# Autodesk Inventor assembly: Сборка2
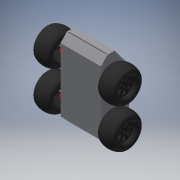
[picture p0: Inventor's stored thumbnail of the model, 180x180]
Saved by Autodesk Inventor 2019 (Build 230136000, 136)
## iProperties
Created: 2022-02-24
Part Number: Сборка2
Material: Типовые
Document SubType Name: Assembly
Designer: korsh
Author: korsh
## Documents named in this file (11)
- C:\Users\korsh\Desktop\Новая папка (7)\Сборка2.iam
- C:\Users\korsh\Desktop\Новая папка (7)\Моторный блок.iam
- C:\Users\korsh\Desktop\Новая папка (7)\боковина.ipt
- C:\Users\korsh\Desktop\Новая папка (7)\дно.ipt
- C:\Users\korsh\Desktop\Новая папка (7)\маленькое дно1.ipt
- C:\Users\korsh\Desktop\Новая папка (7)\мальенькое дно 2.ipt
- C:\Users\korsh\Desktop\Новая папка (7)\Деталь7.ipt
- C:\Users\korsh\Desktop\Новая папка (7)\задняя.ipt
- C:\Users\korsh\Desktop\Новая папка (7)\полуверх.ipt
- C:\Users\korsh\Desktop\Новая папка (7)\полуверх 2.ipt
- C:\Users\korsh\Desktop\Новая папка (7)\верх.ipt
## Components (14 placed, 10 different names)
1. Моторный блок:1 [sub-assembly] — Заподлицо:1, Заподлицо:2, Совмещение:1
2. Моторный блок:2 [sub-assembly] — Заподлицо:1, Заподлицо:2, Совмещение:1, Совмещение:2
3. боковина:1 — Совмещение:2, Заподлицо:3, Заподлицо:4, Совмещение:7, Заподлицо:6, Заподлицо:8, Совмещение:9, Заподлицо:12, Заподлицо:13, Заподлицо:17
4. боковина:2 — Заподлицо:3, Заподлицо:4, Совмещение:3, Совмещение:4, Совмещение:5, Совмещение:6, Совмещение:7, Заподлицо:5, Заподлицо:7, Заподлицо:9, Заподлицо:10, Заподлицо:11, Совмещение:8, Заподлицо:14, Заподлицо:15, Заподлицо:16
5. Моторный блок:3 [sub-assembly] — Совмещение:3, Совмещение:5
6. Моторный блок:4 [sub-assembly] — Совмещение:4, Совмещение:6
7. дно:1 — Заподлицо:5
8. маленькое дно1:1 — Заподлицо:6
9. мальенькое дно 2:1 — Заподлицо:7
10. лицо — Заподлицо:8, Совмещение:9, Заподлицо:12, Заподлицо:13
11. задняя:1 — Заподлицо:9, Заподлицо:10, Заподлицо:11, Совмещение:8
12. полуверх:1 — Заподлицо:14
13. полуверх 2:1 — Заподлицо:15, Заподлицо:16
14. верх:1 — Заподлицо:17
## Relationships (26: Flush 17, Mate 9)
- Заподлицо:1 [Flush]: Моторный блок:1 ↔ Моторный блок:2
- Заподлицо:2 [Flush]: Моторный блок:1 ↔ Моторный блок:2
- Совмещение:1 [Mate] (171 mm): Моторный блок:1 ↔ Моторный блок:2
- Совмещение:2 [Mate]: Моторный блок:2 ↔ боковина:1
- Заподлицо:3 [Flush]: боковина:1 ↔ боковина:2
- Заподлицо:4 [Flush]: боковина:1 ↔ боковина:2
- Совмещение:3 [Mate]: боковина:2 ↔ Моторный блок:3
- Совмещение:4 [Mate]: боковина:2 ↔ Моторный блок:4
- Совмещение:5 [Mate]: боковина:2 ↔ Моторный блок:3
- Совмещение:6 [Mate]: боковина:2 ↔ Моторный блок:4
- Совмещение:7 [Mate] (180 mm): боковина:1 ↔ боковина:2
- Заподлицо:5 [Flush]: боковина:2 ↔ дно:1
- Заподлицо:6 [Flush]: боковина:1 ↔ маленькое дно1:1
- Заподлицо:7 [Flush]: боковина:2 ↔ мальенькое дно 2:1
- Заподлицо:8 [Flush]: боковина:1 ↔ лицо
- Заподлицо:9 [Flush]: боковина:2 ↔ задняя:1
- Заподлицо:10 [Flush]: боковина:2 ↔ задняя:1
- Заподлицо:11 [Flush]: боковина:2 ↔ задняя:1
- Совмещение:8 [Mate]: боковина:2 ↔ задняя:1
- Совмещение:9 [Mate]: боковина:1 ↔ лицо
- Заподлицо:12 [Flush]: боковина:1 ↔ лицо
- Заподлицо:13 [Flush]: боковина:1 ↔ лицо
- Заподлицо:14 [Flush]: боковина:2 ↔ полуверх:1
- Заподлицо:15 [Flush]: боковина:2 ↔ полуверх 2:1
- Заподлицо:16 [Flush]: боковина:2 ↔ полуверх 2:1
- Заподлицо:17 [Flush]: боковина:1 ↔ верх:1
